# Autodesk Inventor assembly: WheelAssembly
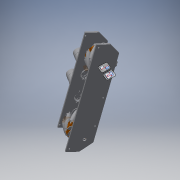
[picture p0: Inventor's stored thumbnail of the model, 180x180]
Saved by Autodesk Inventor 2017 (Build 210142000, 142)
## iProperties
Created: 2016-09-10
Part Number: WheelAssembly
Document SubType Name: Assembly
Designer: RoboticsUser
Author: RoboticsUser
## Documents named in this file (10)
- C:\Robotics\CAD\2016-17_CAD\WheelAssemble2.0-right.iam
- C:\Robotics\CAD\COTSParts\Actobotics\545 parts\545556.ipt
- C:\Robotics\CAD\COTSParts\Actobotics\615 parts\615102.ipt
- C:\Robotics\CAD\COTSParts\Actobotics\634 parts\634080.ipt
- C:\Robotics\CAD\COTSParts\Motors\Andymark 2964  NeveRest 40 Motor.ipt
- C:\Robotics\CAD\COTSParts\Tetrix\tetrix-motor-mounts-1.snapshot.1\Tetrex 2pc motor mount.ipt
- C:\Robotics\CAD\COTSParts\Actobotics\545 parts\545456.ipt
- C:\Robotics\CAD\COTSParts\Wheels\AndyMark Mecanum Wheels\100mm Aluminum Mecanum wheels.ipt
- C:\Robotics\CAD\2016-17_CAD\DrainTrainPlate2.0.iam
- C:\Robotics\CAD\2016-17_CAD\DriveTrainPlate -Inside.ipt
## Components (24 placed, 9 different names)
1. 545556:2 — Mate:73, Mate:74, Mate:75, Mate:76, Mate:77
2. 615102:4 — Mate:35, Mate:36, Mate:37
3. 634080:2 — Insert:100, Mate:77, Mate:79, Mate:81
4. 545556:6 — Insert:83, Mate:46
5. 615102:5 — Mate:44, Mate:46
6. 634080:3 — Mate:28, Mate:30, Mate:44, Mate:50, Insert:95, Insert:96
7. Andymark 2964  NeveRest 40 Motor:2 — Mate:42, Insert:105, Mate:69
8. 545556:8 — Mate:4
9. 545556:9 — Mate:37, Mate:38
10. Andymark 2964  NeveRest 40 Motor:3 — Mate:35, Mate:36, Mate:38, Insert:98, Mate:65, Mate:71, Flush:1
11. Tetrex 2pc motor mount:1 — Mate:69, Mate:70
12. Tetrex 2pc motor mount:2 — Mate:65, Mate:72
13. 545456:1 — Mate:75, Mate:76, Mate:80
14. 545456:3 — Insert:83, Insert:88
15. 615102:6 — Mate:4, Mate:42
16. 615102:7 — Mate:73, Mate:74, Mate:78
17. 100mm Aluminum Mecanum wheels:1 — Insert:88, Mate:27, Mate:50
18. 100mm Aluminum Mecanum wheels:2 — Mate:79, Mate:80, Mate:82
19. 545456:4 — Insert:106, Mate:82
20. 545456:5 — Mate:27, Mate:28, Mate:29
21. 545556:12 — Mate:29, Mate:30, Mate:64
22. 545556:13 — Insert:106, Mate:81
23. DrainTrainPlate2.0:1 [sub-assembly] — Insert:95, Mate:64
24. DriveTrainPlate -Inside:1 — Insert:96, Insert:98, Insert:100, Insert:105, Mate:70, Mate:71, Mate:72, Flush:1, Mate:78
## Relationships (38: Mate 29, Insert 8, Flush 1)
- Insert:83: 545556:6 ↔ 545456:3
- Mate:4: 545556:8 ↔ 615102:6
- Insert:88: 545456:3 ↔ 100mm Aluminum Mecanum wheels:1
- Mate:27: 100mm Aluminum Mecanum wheels:1 ↔ 545456:5
- Mate:28: 634080:3 ↔ 545456:5
- Mate:29: 545456:5 ↔ 545556:12
- Mate:30: 634080:3 ↔ 545556:12
- Mate:35: 615102:4 ↔ Andymark 2964  NeveRest 40 Motor:3
- Mate:36: 615102:4 ↔ Andymark 2964  NeveRest 40 Motor:3
- Mate:37: 615102:4 ↔ 545556:9
- Mate:38: 545556:9 ↔ Andymark 2964  NeveRest 40 Motor:3
- Mate:42: Andymark 2964  NeveRest 40 Motor:2 ↔ 615102:6
- Mate:44: 615102:5 ↔ 634080:3
- Mate:46: 545556:6 ↔ 615102:5
- Mate:50: 634080:3 ↔ 100mm Aluminum Mecanum wheels:1
- Insert:95: 634080:3 ↔ DrainTrainPlate2.0:1
- Mate:64: 545556:12 ↔ DrainTrainPlate2.0:1
- Insert:96: 634080:3 ↔ DriveTrainPlate -Inside:1
- Insert:98: Andymark 2964  NeveRest 40 Motor:3 ↔ DriveTrainPlate -Inside:1
- Insert:100: 634080:2 ↔ DriveTrainPlate -Inside:1
- Mate:65: Andymark 2964  NeveRest 40 Motor:3 ↔ Tetrex 2pc motor mount:2
- Insert:105: Andymark 2964  NeveRest 40 Motor:2 ↔ DriveTrainPlate -Inside:1
- Mate:69: Andymark 2964  NeveRest 40 Motor:2 ↔ Tetrex 2pc motor mount:1
- Mate:70: Tetrex 2pc motor mount:1 ↔ DriveTrainPlate -Inside:1
- Mate:71: Andymark 2964  NeveRest 40 Motor:3 ↔ DriveTrainPlate -Inside:1
- Mate:72: Tetrex 2pc motor mount:2 ↔ DriveTrainPlate -Inside:1
- Flush:1: Andymark 2964  NeveRest 40 Motor:3 ↔ DriveTrainPlate -Inside:1
- Mate:73: 545556:2 ↔ 615102:7
- Mate:74: 545556:2 ↔ 615102:7
- Mate:75: 545556:2 ↔ 545456:1
- Mate:76: 545556:2 ↔ 545456:1
- Mate:77: 545556:2 ↔ 634080:2
- Mate:78 (3.175 mm): 615102:7 ↔ DriveTrainPlate -Inside:1
- Mate:79: 634080:2 ↔ 100mm Aluminum Mecanum wheels:2
- Mate:80: 545456:1 ↔ 100mm Aluminum Mecanum wheels:2
- Insert:106: 545456:4 ↔ 545556:13
- Mate:81: 634080:2 ↔ 545556:13
- Mate:82: 100mm Aluminum Mecanum wheels:2 ↔ 545456:4
